# Autodesk Inventor assembly: BL Motor + Encoder + Gearbox
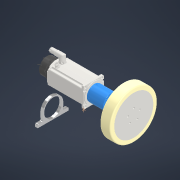
[picture p0: Inventor's stored thumbnail of the model, 180x180]
Saved by Autodesk Inventor 2022 (Build 260153000, 153)
## iProperties
Created: 2021-09-22
Part Number: BL Motor + Encoder + Gearbox
Document SubType Name: Assembly
Designer: seb_0
Author: seb_0
## Documents named in this file (7)
- D:\Documentos\15.PUCP_2021-2\[PDM] Proyecto de Diseño Mecatrónico\ProyectoGIT\ProyectoRobotPallet\Motor\BL Motor + Encoder + Gearbox + Rueda.iam
- D:\Documentos\15.PUCP_2021-2\[PDM] Proyecto de Diseño Mecatrónico\ProyectoGIT\ProyectoRobotPallet\Motor\Encoder - E 600R\e600-8871002100.ipt
- D:\Documentos\15.PUCP_2021-2\[PDM] Proyecto de Diseño Mecatrónico\ProyectoGIT\ProyectoRobotPallet\Motor\Rueda\Rueda.iam
- D:\Documentos\15.PUCP_2021-2\[PDM] Proyecto de Diseño Mecatrónico\ProyectoGIT\ProyectoRobotPallet\Motor\Rueda\Sprocket_Rueda.ipt
- D:\Documentos\15.PUCP_2021-2\[PDM] Proyecto de Diseño Mecatrónico\ProyectoGIT\ProyectoRobotPallet\Motor\BL Motor - BG 95x80 dCore\bg-95x80-885950205312.ipt
- D:\Documentos\15.PUCP_2021-2\[PDM] Proyecto de Diseño Mecatrónico\ProyectoGIT\ProyectoRobotPallet\Motor\Gearbox - PLG 75 HT 10.1\plg-75-8887505053.ipt
- D:\Documentos\15.PUCP_2021-2\[PDM] Proyecto de Diseño Mecatrónico\ProyectoGIT\ProyectoRobotPallet\Soportes\Soporte_Motor_Encoder.ipt
## Components (6 placed, 6 different names)
1. e600-8871002100:1 — Coincidencia:16, Coincidencia:17, Coincidencia:18
2. Rueda:1 [sub-assembly] — Coincidencia:11, Coincidencia:12, Coincidencia:13
3. Sprocket_Rueda:1 — Coincidencia:11, Coincidencia:12, Coincidencia:13, Coincidencia:22, Coincidencia:23, Coincidencia:24
4. bg-95x80-885950205312:1 — Coincidencia:14, Coincidencia:15, Coincidencia:16, Coincidencia:17, Coincidencia:18, Coincidencia:19, Coincidencia:20, Coincidencia:21
5. plg-75-8887505053:1 — Coincidencia:19, Coincidencia:20, Coincidencia:21, Coincidencia:22, Coincidencia:23, Coincidencia:24
6. Soporte_Motor_Encoder:1
## Relationships (14: Mate 14)
- Coincidencia:11 [Mate]: Rueda:1 ↔ Sprocket_Rueda:1
- Coincidencia:12 [Mate]: Rueda:1 ↔ Sprocket_Rueda:1
- Coincidencia:13 [Mate]: Rueda:1 ↔ Sprocket_Rueda:1
- Coincidencia:14 [Mate]: bg-95x80-885950205312:1
- Coincidencia:15 [Mate]: bg-95x80-885950205312:1
- Coincidencia:16 [Mate]: e600-8871002100:1 ↔ bg-95x80-885950205312:1
- Coincidencia:17 [Mate]: e600-8871002100:1 ↔ bg-95x80-885950205312:1
- Coincidencia:18 [Mate]: e600-8871002100:1 ↔ bg-95x80-885950205312:1
- Coincidencia:19 [Mate]: bg-95x80-885950205312:1 ↔ plg-75-8887505053:1
- Coincidencia:20 [Mate]: bg-95x80-885950205312:1 ↔ plg-75-8887505053:1
- Coincidencia:21 [Mate] (-34.858 mm): bg-95x80-885950205312:1 ↔ plg-75-8887505053:1
- Coincidencia:22 [Mate]: Sprocket_Rueda:1 ↔ plg-75-8887505053:1
- Coincidencia:23 [Mate]: Sprocket_Rueda:1 ↔ plg-75-8887505053:1
- Coincidencia:24 [Mate] (5 mm): Sprocket_Rueda:1 ↔ plg-75-8887505053:1
